# Autodesk Inventor assembly: Mont_Mesa1_001
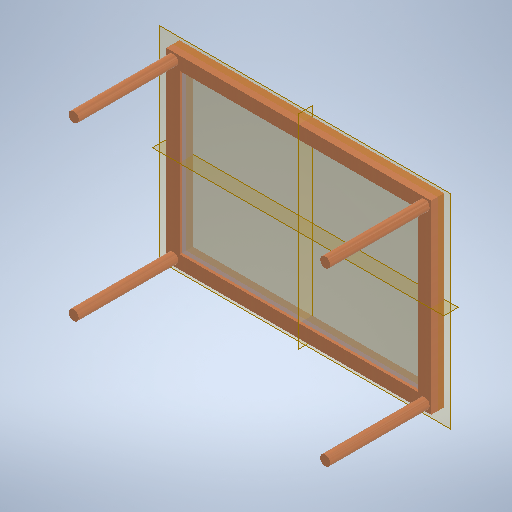
[picture p0: Inventor's stored thumbnail of the model, 512x512]
Saved by Autodesk Inventor 2025.2 (Build 292293000, 293)
## iProperties
Created: 2025-04-07
Part Number: Mont_Mesa1_001
Document SubType Name: Assembly
Designer: Formação
Author: Formação
## Documents named in this file (4)
- C:\Users\Formação\Documents\Inventor\Sessão_25_03_25\Mont_Mesa1_001.iam
- C:\Users\Formação\Documents\Inventor\Sessão_25_03_25\Mesa_001.ipt
- C:\Users\Formação\Documents\Inventor\Sessão_25_03_25\Tampo_vidro.ipt
- C:\Users\Formação\Documents\Inventor\Sessão_25_03_25\Perna_mad_001.ipt
## Components (6 placed, 3 different names)
1. Mesa_001:1 — Alinhado:1, Alinhado:2, Alinhado:3, Alinhado:4, Alinhado:5, Coincidente:1, Coincidente:2
2. Tampo_vidro:1 — Coincidente:1, Alinhado:6, Alinhado:7, Coincidente:2, Coincidente:4
3. Perna_mad_001:1 — Coincidente:4, Coincidente:5, Coincidente:6, Simetria:1, Alinhado:10, Alinhado:11, Simetria:2
4. Perna_mad_001:7 — Coincidente:8, Simetria:2, Alinhado:12, Simetria:3
5. Perna_mad_001:8 — Simetria:1, Alinhado:10, Coincidente:7, Alinhado:11
6. Perna_mad_001:9 — Coincidente:9, Coincidente:10, Coincidente:11, Simetria:3
## Relationships (23: Flush 10, Mate 10, Symmetry 3)
- Alinhado:1 [Flush]: Mesa_001:1
- Alinhado:2 [Flush]: Mesa_001:1
- Alinhado:3 [Flush]: Mesa_001:1
- Alinhado:4 [Flush]: Mesa_001:1
- Alinhado:5 [Flush]: Mesa_001:1
- Coincidente:1 [Mate]: Mesa_001:1 ↔ Tampo_vidro:1
- Alinhado:6 [Flush]: Tampo_vidro:1
- Alinhado:7 [Flush]: Tampo_vidro:1
- Coincidente:2 [Mate]: Mesa_001:1 ↔ Tampo_vidro:1
- Coincidente:4 [Mate]: Tampo_vidro:1 ↔ Perna_mad_001:1
- Coincidente:5 [Mate] (-1620 mm): Perna_mad_001:1
- Coincidente:6 [Mate] (2375.319 mm): Perna_mad_001:1
- Simetria:1 [Symmetry]: Perna_mad_001:1 ↔ Perna_mad_001:8
- Alinhado:10 [Flush]: Perna_mad_001:1 ↔ Perna_mad_001:8
- Coincidente:7 [Mate]: Perna_mad_001:8
- Alinhado:11 [Flush]: Perna_mad_001:1 ↔ Perna_mad_001:8
- Coincidente:8 [Mate]: Perna_mad_001:7
- Simetria:2 [Symmetry]: Perna_mad_001:1 ↔ Perna_mad_001:7
- Coincidente:9 [Mate] (354.186 mm): Perna_mad_001:9
- Coincidente:10 [Mate]: Perna_mad_001:9
- Alinhado:12 [Flush] (1620 mm): Perna_mad_001:7
- Coincidente:11 [Mate] (-2374.457 mm): Perna_mad_001:9
- Simetria:3 [Symmetry]: Perna_mad_001:7 ↔ Perna_mad_001:9
